# Autodesk Inventor assembly: DriveChain2
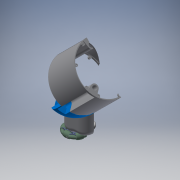
[picture p0: Inventor's stored thumbnail of the model, 180x180]
Saved by Autodesk Inventor 2019.1 (Build 231200000, 200)
## iProperties
Created: 2018-07-27
Part Number: DriveChain2
Material: Generisch
Document SubType Name: Assembly
Designer: JochenAlt
Author: JochenAlt
## Documents named in this file (12)
- D:\Projects\Ondine\CAD\DriveChain.iam
- D:\Projects\Ondine\CAD\Motor.iam
- D:\Projects\Ondine\CAD\HarmonicDrive-Axis.ipt
- D:\Projects\Ondine\CAD\BushOmniWheel.ipt
- D:\Projects\Ondine\CAD\Encoder\Avago Encoder.iam
- D:\Projects\Ondine\CAD\DriveChainEnclosure.ipt
- D:\Projects\Ondine\CAD\BeltDriveAxis.ipt
- D:\Projects\Ondine\CAD\BushBeltDriveTL.ipt
- D:\Projects\Ondine\CAD\Bearings\W 637_4 X-2Z.iam
- D:\Projects\Ondine\CAD\OmniWheel.iam
- D:\Projects\Ondine\CAD\Beltdrive\BeltGear.iam
- D:\Projects\Ondine\CAD\BeltDriveAxisSleeve.ipt
## Components (15 placed, 10 different names)
1. DriveChainEnclosure:1 — Passend:44, Passend:105, Passend:106, Passend:130, Passend:131, Passend:133, Passend:134, Passend:135, Passend:136
2. W 637_4 X-2Z:3 [sub-assembly] — Passend:130, Passend:131
3. W 637_4 X-2Z:2 [sub-assembly]
4. W 637_4 X-2Z:1 [sub-assembly] — Passend:105, Passend:106, Passend:107, Passend:109, Passend:119
5. BushOmniWheel:4 — Passend:82, Passend:119, Passend:128
6. BushOmniWheel:3 — Passend:80
7. BeltdriveAxis — Passend:80, Passend:132, Passend:133, Passend:136, Passend:137, Passend:138
8. Avago Encoder:1 [sub-assembly] — Passend:58, Winkel:1, Passend:113, 10
9. BushOmniWheel:1 — Passend:11, Passend:109, Passend:112
10. HarmonicDrive-Axis:1 — Passend:11, Passend:82, Passend:107, Passend:111, Drehung:8, Passend:125, Passend:126, Drehung:9
11. OmniWheel:1 [sub-assembly] — Passend:111, Drehung:8, Passend:112, Passend:125
12. W 637_4 X-2Z:4 [sub-assembly] — Passend:132, Passend:134, Passend:135
13. NewBeltGear:1 [sub-assembly] — Passend:126, Drehung:9, Passend:128, Passend:129, Passend:137, Passend:139
14. Motor:1 [sub-assembly] — Passend:44, Passend:58, Passend:113, 10, Passend:129
15. BeltDriveAxisSleeve:1 — Passend:138, Passend:139
## Relationships (31: Mate 28, RelateRotation 2, Angle 1)
- Passend:11 [Mate]: BushOmniWheel:1 ↔ HarmonicDrive-Axis:1
- Passend:44 [Mate]: DriveChainEnclosure:1 ↔ Motor:1
- Passend:58 [Mate]: Avago Encoder:1 ↔ Motor:1
- Passend:80 [Mate]: BushOmniWheel:3 ↔ BeltdriveAxis
- Passend:82 [Mate]: BushOmniWheel:4 ↔ HarmonicDrive-Axis:1
- Winkel:1 [Angle] (90 deg): Avago Encoder:1
- Passend:105 [Mate]: DriveChainEnclosure:1 ↔ W 637_4 X-2Z:1
- Passend:106 [Mate]: DriveChainEnclosure:1 ↔ W 637_4 X-2Z:1
- Passend:107 [Mate]: W 637_4 X-2Z:1 ↔ HarmonicDrive-Axis:1
- Passend:109 [Mate]: W 637_4 X-2Z:1 ↔ BushOmniWheel:1
- Passend:111 [Mate]: HarmonicDrive-Axis:1 ↔ OmniWheel:1
- Drehung:8 [RelateRotation] (1 ul): HarmonicDrive-Axis:1 ↔ OmniWheel:1
- Passend:112 [Mate]: BushOmniWheel:1 ↔ OmniWheel:1
- Passend:113 [Mate]: Avago Encoder:1 ↔ Motor:1
- 10 [Mate]: Avago Encoder:1 ↔ Motor:1
- Passend:119 [Mate]: W 637_4 X-2Z:1 ↔ BushOmniWheel:4
- Passend:125 [Mate]: HarmonicDrive-Axis:1 ↔ OmniWheel:1
- Passend:126 [Mate]: HarmonicDrive-Axis:1 ↔ NewBeltGear:1
- Drehung:9 [RelateRotation] (1 ul): HarmonicDrive-Axis:1 ↔ NewBeltGear:1
- Passend:128 [Mate]: BushOmniWheel:4 ↔ NewBeltGear:1
- Passend:129 [Mate] (0.5 mm): NewBeltGear:1 ↔ Motor:1
- Passend:130 [Mate]: DriveChainEnclosure:1 ↔ W 637_4 X-2Z:3
- Passend:131 [Mate]: DriveChainEnclosure:1 ↔ W 637_4 X-2Z:3
- Passend:132 [Mate]: BeltdriveAxis ↔ W 637_4 X-2Z:4
- Passend:133 [Mate]: DriveChainEnclosure:1 ↔ BeltdriveAxis
- Passend:134 [Mate]: DriveChainEnclosure:1 ↔ W 637_4 X-2Z:4
- Passend:135 [Mate]: DriveChainEnclosure:1 ↔ W 637_4 X-2Z:4
- Passend:136 [Mate]: DriveChainEnclosure:1 ↔ BeltdriveAxis
- Passend:137 [Mate]: BeltdriveAxis ↔ NewBeltGear:1
- Passend:138 [Mate]: BeltdriveAxis ↔ BeltDriveAxisSleeve:1
- Passend:139 [Mate]: NewBeltGear:1 ↔ BeltDriveAxisSleeve:1
